# Autodesk Inventor assembly: BUILDINGINV
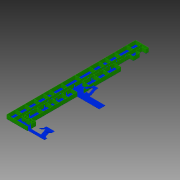
[picture p0: Inventor's stored thumbnail of the model, 180x180]
Saved by Autodesk Inventor 2013 SP2 (Build 170200200, 200)
## iProperties
Created: 2015-01-19
Part Number: BUILDINGINV
Document SubType Name: Assembly
Designer: Working
Author: Working
## Documents named in this file (3)
- D:\onedrive\文档\inventor\机电楼三维模型\BUILDINGINV.iam
- D:\onedrive\文档\inventor\机电楼三维模型\ipt\4-D-地.ipt
- D:\onedrive\文档\inventor\机电楼三维模型\ipt\4-D-墙.ipt
## Components (2 placed, 2 different names)
1. 4-D-地:1 — 表面齐平:1, 表面齐平:2, 配合:1, 表面齐平:3, 表面齐平:4, 配合:2
2. 4-D-墙:1 — 表面齐平:3, 表面齐平:4, 配合:2
## Relationships (6: Flush 4, Mate 2)
- 表面齐平:1 [Flush]: 4-D-地:1
- 表面齐平:2 [Flush]: 4-D-地:1
- 配合:1 [Mate]: 4-D-地:1
- 表面齐平:3 [Flush]: 4-D-地:1 ↔ 4-D-墙:1
- 表面齐平:4 [Flush]: 4-D-地:1 ↔ 4-D-墙:1
- 配合:2 [Mate]: 4-D-地:1 ↔ 4-D-墙:1
